# Autodesk Inventor assembly: Assembly15
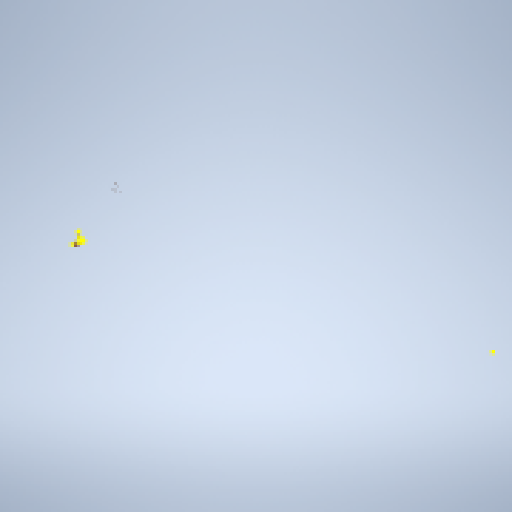
[picture p0: Inventor's stored thumbnail of the model, 512x512]
Saved by Autodesk Inventor 2024.1 (Build 281209000, 209)
## iProperties
Created: 2023-11-10
Part Number: Assembly15
Document SubType Name: Assembly
Designer: luvag
Author: luvag
## Documents named in this file (3)
- C:\Users\luvag\Desktop\Assembly15.iam
- C:\Users\luvag\Desktop\Assembly14.iam
- C:\Users\luvag\Desktop\sid ga.ipt
## Components (2 placed, 2 different names)
1. Assembly14:1 [sub-assembly]
2. sid ga:1
## Relationships (1: WeldJoint 1)
- [WeldJoint]: Assembly14:1 ↔ sid ga:1
